# Autodesk Inventor assembly: Assembly312
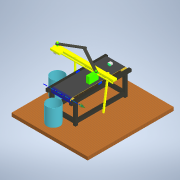
[picture p0: Inventor's stored thumbnail of the model, 180x180]
Saved by Autodesk Inventor 2022 (Build 260153000, 153)
## iProperties
Created: 2021-07-14
Part Number: Assembly312
Document SubType Name: Assembly
Designer: sachin
Author: sachin
## Documents named in this file (14)
- C:\Users\DELL\Downloads\Assembly312 (5).iam
- C:\Users\DELL\Downloads\Traka.ipt
- C:\Users\DELL\Downloads\box.ipt
- C:\Users\DELL\Downloads\platformm.ipt
- C:\Users\DELL\Downloads\crank part.ipt
- C:\Users\DELL\Downloads\new bolt.ipt
- C:\Users\DELL\Downloads\new slider part.ipt
- C:\Users\DELL\Downloads\new slider.ipt
- C:\Users\DELL\Downloads\cranker rod part.ipt
- C:\Users\DELL\Downloads\container 2 (1).ipt
- F:\pillar.ipt
- F:\canon\ur sensor.ipt
- F:\fianl box.ipt
- F:\box.ipt
## Components (17 placed, 12 different names)
1. Traka:1 — Mate:20, Flush:15, Mate:29, Flush:18, Mate:30
2. platformm:2 — Mate:20, Flush:15, Mate:28, Mate:31
3. new bolt:1 — Rotational:1, Mate:25, Mate:27
4. new slider:1 — Rotational:1, Rotational:2
5. cranker rod part:2 — Mate:23, Mate:24, Mate:26
6. crank part:2 — Rotational:2, Mate:23, Mate:24
7. new slider part:1 — Mate:25, Mate:26, Mate:27, Mate:32
8. container 2 (1):1 — Mate:28
9. box:1 — Mate:29, Flush:18, Mate:30
10. container 2 (1):2 — Mate:31
11. pillar:1
12. pillar:2
13. ur sensor:1
14. ur sensor:2
15. ur sensor:3
16. fianl box:1
17. box:2 — Mate:32
## Relationships (15: Mate 11, Flush 2, RevoluteJoint 2)
- Mate:20: Traka:1 ↔ platformm:2
- Flush:15 (76.2 mm): Traka:1 ↔ platformm:2
- Rotational:1 [RevoluteJoint]: new bolt:1 ↔ new slider:1
- Rotational:2 [RevoluteJoint] (-10.16 mm): new slider:1 ↔ crank part:2
- Mate:23: cranker rod part:2 ↔ crank part:2
- Mate:24: cranker rod part:2 ↔ crank part:2
- Mate:25: new bolt:1 ↔ new slider part:1
- Mate:26: cranker rod part:2 ↔ new slider part:1
- Mate:27 (254 mm): new bolt:1 ↔ new slider part:1
- Mate:28: platformm:2 ↔ container 2 (1):1
- Mate:29: Traka:1 ↔ box:1
- Flush:18 (63.5 mm): Traka:1 ↔ box:1
- Mate:30 (355.6 mm): Traka:1 ↔ box:1
- Mate:31: platformm:2 ↔ container 2 (1):2
- Mate:32: new slider part:1 ↔ box:2
